# Autodesk Inventor assembly: assembly
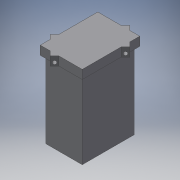
[picture p0: Inventor's stored thumbnail of the model, 180x180]
Saved by Autodesk Inventor 2019 (Build 230136000, 136)
## iProperties
Created: 2021-05-02
Part Number: assembly
Material: Generisch
Document SubType Name: Assembly
Designer: Michael Hohenstein
Author: Michael Hohenstein
## Documents named in this file (3)
- C:\Users\Michael Hohenstein\Desktop\Github\Plant\case\assembly.iam
- C:\Users\Michael Hohenstein\Desktop\Github\Plant\case\cage.ipt
- C:\Users\Michael Hohenstein\Desktop\Github\Plant\case\lid.ipt
## Components (2 placed, 2 different names)
1. cage:1 — Passend:2, Passend:3, Passend:4
2. lid:1 — Passend:2, Passend:3, Passend:4
## Relationships (3: Mate 3)
- Passend:2 [Mate] (0.25 mm): cage:1 ↔ lid:1
- Passend:3 [Mate] (0.25 mm): cage:1 ↔ lid:1
- Passend:4 [Mate] (0.25 mm): cage:1 ↔ lid:1
